# Autodesk Inventor assembly: HIP_UNIT
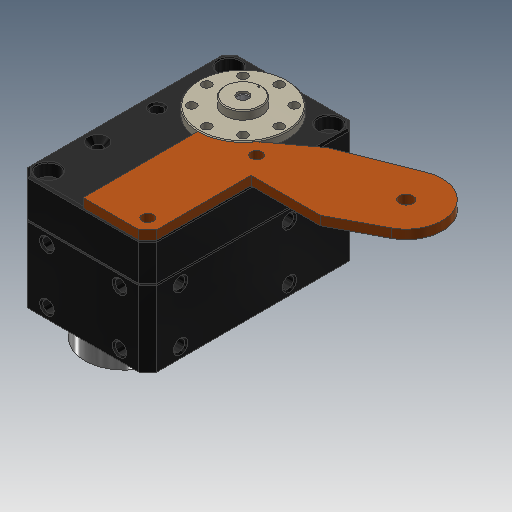
[picture p0: Inventor's stored thumbnail of the model, 512x512]
Saved by Autodesk Inventor 2019.4 (Build 234330000, 330)
## iProperties
Created: 2019-11-06
Part Number: HIP_UNIT
Material: 一般
Document SubType Name: Assembly
Designer: y6tada
Author: y6tada
## Documents named in this file (3)
- C:\Workspace\Yuni9\Inventor\Asm\HIP_UNIT\HIP_UNIT.iam
- C:\Workspace\Yuni9\Inventor\Libs\DYNAMIXEL\XM430\XM430_ASM_WITHOUT-BACK.iam
- C:\Workspace\Yuni9\Inventor\Asm\HIP_UNIT\HIP_TOPFRAME2.ipt
## Components (2 placed, 2 different names)
1. XM430_ASM_WITHOUT-BACK:1 [sub-assembly] — フラッシュ:1
2. HIP_TOPFRAME2:1 — フラッシュ:1
## Relationships (1: Flush 1)
- フラッシュ:1 [Flush]: XM430_ASM_WITHOUT-BACK:1 ↔ HIP_TOPFRAME2:1
